# Autodesk Inventor assembly: 30-Translational
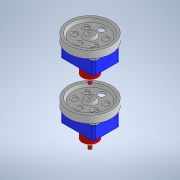
[picture p0: Inventor's stored thumbnail of the model, 180x180]
Saved by Autodesk Inventor 2022 (Build 260153000, 153)
## iProperties
Created: 2022-08-14
Part Number: 30-Translational
Document SubType Name: Assembly
Designer: Nick
Mass: 374.596 g
Surface Area: 784.562 cm^2
Volume: 223.032 cm^3
Density: 1.67957 g/cm^3
Author: Nick
## Documents named in this file (6)
- Y:\Projects\BattleBot\30-Translational.iam
- Y:\Projects\BattleBot\Motor.ipt
- Y:\Projects\BattleBot\Gearbox.ipt
- Y:\Projects\BattleBot\Gearbox Mount.ipt
- Y:\Projects\BattleBot\Wheel.ipt
- Y:\Projects\BattleBot\Gearbox Outer Mount.ipt
## Components (10 placed, 5 different names)
1. Motor:1 — Insert:2, Angle:1
2. Gearbox:1 — Insert:1, Insert:3, Insert:4
3. Gearbox Mount:1 — Insert:1, Insert:2, Flush:1, Angle:1
4. Wheel:1 — Insert:3
5. Gearbox Outer Mount:1 — Insert:4, Flush:1
6. Motor:2
7. Gearbox:2
8. Gearbox Mount:2
9. Wheel:2
10. Gearbox Outer Mount:2
## Component patterns: (2 elements, first: Motor:1 + Gearbox:1 + Gearbox Mount:1 + Wheel:1 + Gearbox Outer Mount:1)
## Relationships (6: Insert 4, Flush 1, Angle 1)
- Insert:1: Gearbox:1 ↔ Gearbox Mount:1
- Insert:2: Motor:1 ↔ Gearbox Mount:1
- Insert:3: Gearbox:1 ↔ Wheel:1
- Insert:4: Gearbox:1 ↔ Gearbox Outer Mount:1
- Flush:1: Gearbox Mount:1 ↔ Gearbox Outer Mount:1
- Angle:1 (0 deg): Motor:1 ↔ Gearbox Mount:1
